# Autodesk Inventor assembly: flyporter_combinations
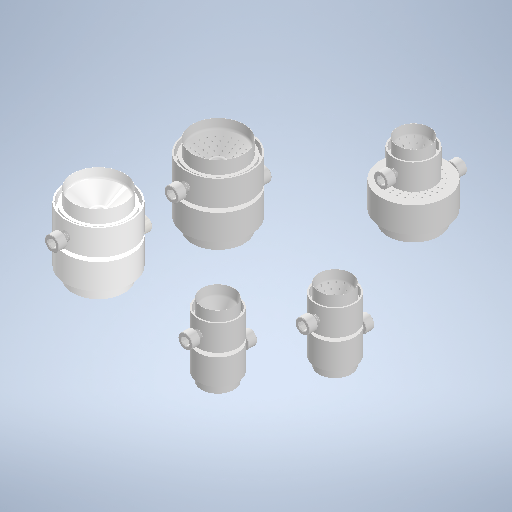
[picture p0: Inventor's stored thumbnail of the model, 512x512]
Saved by Autodesk Inventor 2025 (Build 290162010, 162A)
## iProperties
Created: 2025-04-24
Part Number: flyporter_combinations
Document SubType Name: Assembly
Designer: dinesh
Author: dinesh
## iProperties of the stored document M6_30mm_91290A332_Alloy_steel.ipt
Company: Managed by Terraform
Created: 2023-01-11
Part Number: 91290A332_Alloy Steel Socket Head Screw
Material: Generic
Description: STEP AP203
Document SubType Name: Modeling
Designer: dinesh
Density: 1 g/cm^3
Appearance: Default
Sending System: SolidWorks 2017
Preprocessor: SwSTEP 2.0
Title: 91290A332_Alloy Steel Socket Head Screw.STEP
Author: Administrator
Revision Number: ANY
## iProperties of the stored document M6_20mm_91290A326_Alloy_steel.ipt
Company: Managed by Terraform
Created: 2023-01-11
Part Number: 91290A326_Alloy Steel Socket Head Screw
Material: Generic
Description: STEP AP203
Document SubType Name: Modeling
Designer: dinesh
Density: 1 g/cm^3
Appearance: Default
Sending System: SolidWorks 2017
Preprocessor: SwSTEP 2.0
Title: 91290A326_Alloy Steel Socket Head Screw.STEP
Author: Administrator
Revision Number: ANY
## iProperties of the stored document mcmaster_94669A175_M6_Spacer.ipt
Company: Managed by Terraform
Created: 2025-01-27
Part Number: 94669A175_Aluminum Unthreaded Spacer
Material: Generic
Description: STEP AP203
Document SubType Name: Modeling
Designer: dinesh
Density: 1 g/cm^3
Appearance: Default
Sending System: SolidWorks 2017
Preprocessor: SwSTEP 2.0
Title: 94669A175_Aluminum Unthreaded Spacer.STEP
Author: Administrator
Revision Number: ANY
## Documents named in this file (11)
- C:\Users\dinesh\Documents\GitHub\flytools\flyporter\flyporter_combinations.iam
- C:\Users\dinesh\Documents\GitHub\flytools\flyporter\bottle\flyport_bottle.ipt
- **C:\Users\dinesh\Documents\GitHub\flytools\flyporter\flyporter_combinations.iam*LocalDocs*xAaaaqldaAaaaaaaaAaaaaf3tAf*mcmaster_94669A175_M6_Spacer.ipt
- **C:\Users\dinesh\Documents\GitHub\flytools\flyporter\flyporter_combinations.iam*LocalDocs*xAaaaq3daAaaaaaaaAaaaajmjOf*M6_30mm_91290A332_Alloy_steel.ipt
- C:\Users\dinesh\Documents\GitHub\flytools\flyporter\bottle\perforated_flyport_bottle.ipt
- C:\Users\dinesh\Documents\GitHub\flytools\flyporter\vial\flyport_vial.ipt
- **C:\Users\dinesh\Documents\GitHub\flytools\flyporter\flyporter_combinations.iam*LocalDocs*xAaaaabbaAaaaaaaaAaaaq1kcWh*M6_20mm_91290A326_Alloy_steel.ipt
- C:\Users\dinesh\Documents\GitHub\flytools\flyporter\vial\perforated_flyport_vial.ipt
- C:\Users\dinesh\Documents\GitHub\flytools\flyporter\adapter\mcmaster_94669A175_M6_Spacer.STEP
- C:\Users\dinesh\Documents\GitHub\flytools\flyporter\screws\M6_30mm_91290A332_Alloy_steel.STEP
- C:\Users\dinesh\Documents\GitHub\flytools\flyporter\screws\M6_20mm_91290A326_Alloy_steel.STEP
## Components (25 placed, 7 different names)
1. flyport_bottle:1 — Mate:1, Mate:2, Mate:3, Mate:4
2. mcmaster_94669A175_M6_Spacer:1 — Mate:1, Mate:2, Mate:9
3. M6_30mm_91290A332_Alloy_steel:1 — Mate:3, Mate:4
4. flyport_bottle:2 — Mate:9
5. M6_30mm_91290A332_Alloy_steel:2
6. perforated_flyport_bottle:2
7. mcmaster_94669A175_M6_Spacer:2
8. M6_30mm_91290A332_Alloy_steel:3
9. perforated_flyport_bottle:1
10. M6_30mm_91290A332_Alloy_steel:4
11. flyport_vial:1 — Mate:17, Mate:18, Mate:19, Mate:20
12. mcmaster_94669A175_M6_Spacer:3 — Mate:17, Mate:18, Mate:25
13. M6_20mm_91290A326_Alloy_steel:1 — Mate:19, Mate:20
14. flyport_vial:2 — Mate:25
15. M6_20mm_91290A326_Alloy_steel:2
16. perforated_flyport_vial:2
17. mcmaster_94669A175_M6_Spacer:4
18. M6_20mm_91290A326_Alloy_steel:3
19. perforated_flyport_vial:1
20. M6_20mm_91290A326_Alloy_steel:4
21. perforated_flyport_bottle:3
22. mcmaster_94669A175_M6_Spacer:5 — Mate:39
23. M6_30mm_91290A332_Alloy_steel:5
24. perforated_flyport_vial:3 — Mate:39
25. M6_20mm_91290A326_Alloy_steel:5
## Relationships (35: Mate 35)
- Mate:1: flyport_bottle:1 ↔ mcmaster_94669A175_M6_Spacer:1
- Mate:2: flyport_bottle:1 ↔ mcmaster_94669A175_M6_Spacer:1
- Mate:3: flyport_bottle:1 ↔ M6_30mm_91290A332_Alloy_steel:1
- Mate:4: flyport_bottle:1 ↔ M6_30mm_91290A332_Alloy_steel:1
- [Mate]: flyport_bottle:2 ↔ M6_30mm_91290A332_Alloy_steel:2
- [Mate]: flyport_bottle:2 ↔ M6_30mm_91290A332_Alloy_steel:2
- Mate:9: mcmaster_94669A175_M6_Spacer:1 ↔ flyport_bottle:2
- [Mate]: perforated_flyport_bottle:2 ↔ mcmaster_94669A175_M6_Spacer:2
- [Mate]: perforated_flyport_bottle:2 ↔ mcmaster_94669A175_M6_Spacer:2
- [Mate]: perforated_flyport_bottle:2 ↔ M6_30mm_91290A332_Alloy_steel:3
- [Mate]: perforated_flyport_bottle:2 ↔ M6_30mm_91290A332_Alloy_steel:3
- [Mate]: perforated_flyport_bottle:1 ↔ M6_30mm_91290A332_Alloy_steel:4
- [Mate]: perforated_flyport_bottle:1 ↔ M6_30mm_91290A332_Alloy_steel:4
- [Mate]: mcmaster_94669A175_M6_Spacer:2 ↔ perforated_flyport_bottle:1
- Mate:17: flyport_vial:1 ↔ mcmaster_94669A175_M6_Spacer:3
- Mate:18: flyport_vial:1 ↔ mcmaster_94669A175_M6_Spacer:3
- Mate:19: flyport_vial:1 ↔ M6_20mm_91290A326_Alloy_steel:1
- Mate:20: flyport_vial:1 ↔ M6_20mm_91290A326_Alloy_steel:1
- [Mate]: flyport_vial:2 ↔ M6_20mm_91290A326_Alloy_steel:2
- [Mate]: flyport_vial:2 ↔ M6_20mm_91290A326_Alloy_steel:2
- Mate:25: mcmaster_94669A175_M6_Spacer:3 ↔ flyport_vial:2
- [Mate]: perforated_flyport_vial:2 ↔ mcmaster_94669A175_M6_Spacer:4
- [Mate]: perforated_flyport_vial:2 ↔ mcmaster_94669A175_M6_Spacer:4
- [Mate]: perforated_flyport_vial:2 ↔ M6_20mm_91290A326_Alloy_steel:3
- [Mate]: perforated_flyport_vial:2 ↔ M6_20mm_91290A326_Alloy_steel:3
- [Mate]: perforated_flyport_vial:1 ↔ M6_20mm_91290A326_Alloy_steel:4
- [Mate]: perforated_flyport_vial:1 ↔ M6_20mm_91290A326_Alloy_steel:4
- [Mate]: mcmaster_94669A175_M6_Spacer:4 ↔ perforated_flyport_vial:1
- [Mate]: perforated_flyport_bottle:3 ↔ mcmaster_94669A175_M6_Spacer:5
- [Mate]: perforated_flyport_bottle:3 ↔ mcmaster_94669A175_M6_Spacer:5
- [Mate]: perforated_flyport_bottle:3 ↔ M6_30mm_91290A332_Alloy_steel:5
- [Mate]: perforated_flyport_bottle:3 ↔ M6_30mm_91290A332_Alloy_steel:5
- [Mate]: perforated_flyport_vial:3 ↔ M6_20mm_91290A326_Alloy_steel:5
- [Mate]: perforated_flyport_vial:3 ↔ M6_20mm_91290A326_Alloy_steel:5
- Mate:39: mcmaster_94669A175_M6_Spacer:5 ↔ perforated_flyport_vial:3
## Named parameters: d9_d5 = 0 mm, d10_d6 = 0 mm, d12_d0 = 0 mm, d13_d1 = 0 mm, d14_d5 = 0 mm, d15_d6 = 0 mm, d16_d9_d5 = 0 mm, d17_d10_d6 = 0 mm, d18_d11 = 0 mm, d34_d30 = 0 mm, d35_d31 = 0 mm, d37_d26 = 0 mm, d38_d27 = 0 mm, d39_d30 = 0 mm, d40_d31 = 0 mm, d41_d34_d30 = 0 mm, d42_d35_d31 = 0 mm, d43_d36 = 0 mm, d44_d12_d0 = 0 mm, d45_d13_d1 = 0 mm, d46_d14_d5 = 0 mm, d47_d15_d6 = 0 mm, d51_d41_d34_d30 = 0 mm, d52_d42_d35_d31 = 0 mm
